# Autodesk Inventor assembly: UBG_Nema_17
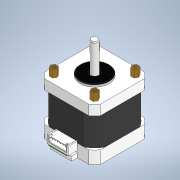
[picture p0: Inventor's stored thumbnail of the model, 180x180]
Saved by Autodesk Inventor 2022.2 (Build 262287010, 287A)
## iProperties
Created: 2022-05-02
Part Number: UBG_Nema_17
Document SubType Name: Assembly
Designer: MXBD
Author: MXBD
## Documents named in this file (3)
- D:\Laser_Engraver\CAD\Assemblies\UBG_Nema_17.iam
- D:\Laser_Engraver\CAD\Parts\03_NEMA17_Motor_45Ncm.ipt
- D:\Laser_Engraver\CAD\Parts\22_Hexnut_5mm.ipt
## Components (5 placed, 2 different names)
1. 03_NEMA17_Motor_45Ncm:1 — Passend:1, Passend:2, Passend:3, Passend:4, Passend:5, Passend:6, Passend:7, Passend:8, Winkel:1, Winkel:2, Winkel:3, Winkel:4
2. 22_Hexnut_5mm:1 — Passend:4, Passend:5, Winkel:3
3. 22_Hexnut_5mm:2 — Passend:3, Passend:6, Winkel:2
4. 22_Hexnut_5mm:3 — Passend:2, Passend:7, Winkel:1
5. 22_Hexnut_5mm:4 — Passend:1, Passend:8, Winkel:4
## Relationships (12: Mate 8, Angle 4)
- Passend:1 [Mate]: 03_NEMA17_Motor_45Ncm:1 ↔ 22_Hexnut_5mm:4
- Passend:2 [Mate]: 03_NEMA17_Motor_45Ncm:1 ↔ 22_Hexnut_5mm:3
- Passend:3 [Mate]: 03_NEMA17_Motor_45Ncm:1 ↔ 22_Hexnut_5mm:2
- Passend:4 [Mate]: 03_NEMA17_Motor_45Ncm:1 ↔ 22_Hexnut_5mm:1
- Passend:5 [Mate]: 03_NEMA17_Motor_45Ncm:1 ↔ 22_Hexnut_5mm:1
- Passend:6 [Mate]: 03_NEMA17_Motor_45Ncm:1 ↔ 22_Hexnut_5mm:2
- Passend:7 [Mate]: 03_NEMA17_Motor_45Ncm:1 ↔ 22_Hexnut_5mm:3
- Passend:8 [Mate]: 03_NEMA17_Motor_45Ncm:1 ↔ 22_Hexnut_5mm:4
- Winkel:1 [Angle] (0 deg): 03_NEMA17_Motor_45Ncm:1 ↔ 22_Hexnut_5mm:3
- Winkel:2 [Angle] (0 deg): 03_NEMA17_Motor_45Ncm:1 ↔ 22_Hexnut_5mm:2
- Winkel:3 [Angle] (0 deg): 03_NEMA17_Motor_45Ncm:1 ↔ 22_Hexnut_5mm:1
- Winkel:4 [Angle] (0 deg): 03_NEMA17_Motor_45Ncm:1 ↔ 22_Hexnut_5mm:4
